# Autodesk Inventor assembly: White King
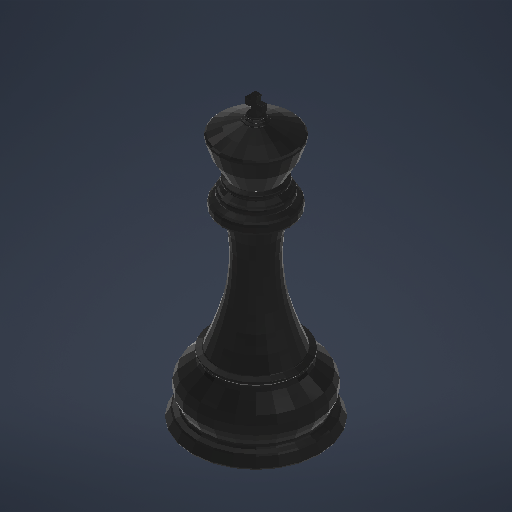
[picture p0: Inventor's stored thumbnail of the model, 512x512]
Saved by Autodesk Inventor 2026 (Build 300175000, 175)
## iProperties
Created: 2025-04-17
Part Number: White King
Document SubType Name: Assembly
Designer: ckyiu
Author: ckyiu
## Documents named in this file (4)
- C:\Users\ckyiu\Documents\Projects\Chessboard-Design\Assemblies\Chess Pieces\Black King.iam
- C:\Users\ckyiu\Documents\Projects\Chessboard-Design\Parts\Chess Pieces\White King Body.ipt
- C:\Users\ckyiu\Documents\Projects\Chessboard-Design\Parts\Generic Neodynium Magnet 10mm diameter 2mm height.ipt
- C:\Users\ckyiu\Documents\Projects\Chessboard-Design\Parts\Chess Pieces\White King Head.ipt
## Components (3 placed, 3 different names)
1. White King Body:1 — Insert:1, Mate:1, Mate:2, Mate:3
2. Generic Neodynium Magnet 10mm diameter 2mm height:1 — Insert:1
3. White King Head:1 — Mate:1, Mate:2, Mate:3
## Relationships (4: Mate 3, Insert 1)
- Insert:1: White King Body:1 ↔ Generic Neodynium Magnet 10mm diameter 2mm height:1
- Mate:1 (0.2 mm): White King Body:1 ↔ White King Head:1
- Mate:2 (0.2 mm): White King Body:1 ↔ White King Head:1
- Mate:3 (0.2 mm): White King Body:1 ↔ White King Head:1
